# Autodesk Inventor assembly: Intake
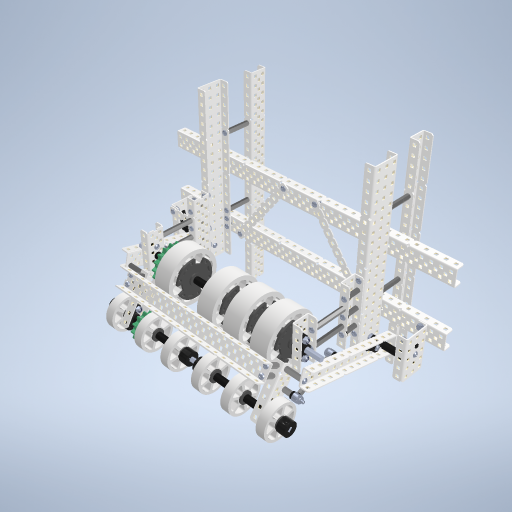
[picture p0: Inventor's stored thumbnail of the model, 512x512]
Saved by Autodesk Inventor 2023 (Build 270158000, 158)
## iProperties
Created: 2022-09-02
Part Number: Intake
Document SubType Name: Assembly
Designer: alex
Author: alex
## Documents named in this file (42)
- C:\Users\alex\Documents\GitHub\4067X_spin_up_cad\Mechanism\Intake.iam
- C:\Users\alex\Documents\GitHub\4067X_spin_up_cad\Library\Structure\Standoff\Standoff 1.00.ipt
- C:\Users\alex\Documents\GitHub\4067X_spin_up_cad\Library\Structure\Standoff.ipt
- C:\Users\alex\Documents\GitHub\4067X_spin_up_cad\Library\Structure\Hardware\Screw Steel - Star\SScrew Star Smooth .290.ipt
- C:\Users\alex\Documents\GitHub\4067X_spin_up_cad\Library\Structure\Hardware\Screw Steel - Star.ipt
- C:\Users\alex\Documents\GitHub\4067X_spin_up_cad\Library\Structure\Standoff\Standoff .50.ipt
- C:\Users\alex\Documents\GitHub\4067X_spin_up_cad\Library\Motion\Spacers\Spacer Nylon .375 OD.ipt
- C:\Users\alex\Documents\GitHub\4067X_spin_up_cad\Library\Structure\Hardware\Nut Keps.ipt
- C:\Users\alex\Documents\GitHub\4067X_spin_up_cad\Library\Motion\1-Post Bearing Flat Hex Retainer.ipt
- C:\Users\alex\Documents\GitHub\4067X_spin_up_cad\Library\Structure\Hardware\Screw Steel - Star\SScrew Star Smooth .375.ipt
- C:\Users\alex\Documents\GitHub\4067X_spin_up_cad\Library\Structure\Hardware\Nut Nylock.ipt
- C:\Users\alex\Documents\GitHub\4067X_spin_up_cad\Library\Structure\C-Channels\Aluminum 1x3x1\Alu C 1x3x1x20.ipt
- C:\Users\alex\Documents\GitHub\4067X_spin_up_cad\Library\Structure\C-Channels\Aluminum 1x3x1\Alu C 1x3x1x5.ipt
- C:\Users\alex\Documents\GitHub\4067X_spin_up_cad\Library\Structure\C-Channels\Aluminum 1x2x1\Alu C 1x2x1x35.ipt
- C:\Users\alex\Documents\GitHub\4067X_spin_up_cad\Library\Structure\Hardware\Screw Steel - Star\SScrew Star Smooth 2.500.ipt
- C:\Users\alex\Documents\GitHub\4067X_spin_up_cad\Library\Motion\Spacers\Spacer Nylon .375 OD\NSpacer .375 OD x .375.ipt
- C:\Users\alex\Documents\GitHub\4067X_spin_up_cad\Library\Motion\Spacers\Spacer Nylon .375 OD\NSpacer .375 OD x .500.ipt
- C:\Users\alex\Documents\GitHub\4067X_spin_up_cad\Library\Structure\C-Channels\Aluminum 1x2x1\Alu C 1x2x1x25.ipt
- C:\Users\alex\Documents\GitHub\4067X_spin_up_cad\Library\Structure\Hardware\Screw Steel - Star\SScrew Star Smooth .750.ipt
- C:\Users\alex\Documents\GitHub\4067X_spin_up_cad\Mechanism\FloatingIntake.iam
- C:\Users\alex\Documents\GitHub\4067X_spin_up_cad\Library\Motion\Spacers\Spacer Nylon .375 OD\NSpacer .375 OD x .250.ipt
- C:\Users\alex\Documents\GitHub\4067X_spin_up_cad\Library\Motion\Spacers\Washer Teflon\TWasher .375 OD x .06250.ipt
- C:\Users\alex\Documents\GitHub\4067X_spin_up_cad\Library\Motion\Spacers\Washer Teflon.ipt
- C:\Users\alex\Documents\GitHub\4067X_spin_up_cad\Library\Motion\Spacers\Washer Teflon\TWasher .375 OD x .04000.ipt
- C:\Users\alex\Documents\GitHub\4067X_spin_up_cad\Library\Structure\Plates\Aluminum\VEX Plates\Alu Plate VEX 1x11.ipt
- C:\Users\alex\Documents\GitHub\4067X_spin_up_cad\Library\Structure\Plates\Aluminum\VEX Plates\Alu Plate VEX 1x6.ipt
- C:\Users\alex\Documents\GitHub\4067X_spin_up_cad\Library\Structure\Standoff\Standoff 2.00.ipt
- C:\Users\alex\Documents\GitHub\4067X_spin_up_cad\Library\Structure\C-Channels\Aluminum 1x2x1\Alu C 1x2x1x5.ipt
- C:\Users\alex\Documents\GitHub\4067X_spin_up_cad\Library\Structure\C-Channels\Aluminum 1x2x1\Alu C 1x2x1x7.ipt
- C:\Users\alex\Documents\GitHub\4067X_spin_up_cad\Library\Structure\Standoff\Standoff .75.ipt
- C:\Users\alex\Documents\GitHub\4067X_spin_up_cad\Library\Motion\Spacers\Spacer Nylon .375 OD\NSpacer .375 OD x .125.ipt
- C:\Users\alex\Documents\GitHub\4067X_spin_up_cad\Library\Motion\Shaft HS\HS Bearing Flat.ipt
- C:\Users\alex\Documents\GitHub\4067X_spin_up_cad\Library\Structure\Hardware\Nut Thin Nylock.ipt
- C:\Users\alex\Documents\GitHub\4067X_spin_up_cad\Library\Structure\Hardware\Screw Steel - Star\SScrew Star Smooth .500.ipt
- C:\Users\alex\Documents\GitHub\4067X_spin_up_cad\Library\Motion\Shaft HS\Shaft HS\Shaft HS 12.0 in.ipt
- C:\Users\alex\Documents\GitHub\4067X_spin_up_cad\Library\Motion\Shaft HS\Shaft HS.ipt
- C:\Users\alex\Documents\GitHub\4067X_spin_up_cad\Library\Motion\Shaft HS\HS Spacer.ipt
- C:\Users\alex\Documents\GitHub\4067X_spin_up_cad\Library\3FlexWheel.iam
- C:\Users\alex\Documents\GitHub\4067X_spin_up_cad\Library\Motion\Shaft HS\HS Spacer\HSpacer .2500.ipt
- C:\Users\alex\Documents\GitHub\4067X_spin_up_cad\Library\Motion\Shaft HS\HS Spacer\HSpacer .5000.ipt
- C:\Users\alex\Documents\GitHub\4067X_spin_up_cad\Library\Motion\Sprockets\HS 18T Sprocket, No Insert.ipt
- C:\Users\alex\Documents\GitHub\4067X_spin_up_cad\Library\Motion\Shaft HS\HS Spacer\HSpacer .1250.ipt
## Components (148 placed, 35 different names)
1. Alu C 1x3x1x5:1 — Insert:107, Insert:108, Insert:120, Mate:15, Insert:145, Insert:230, Insert:244, Insert:245
2. Alu C 1x2x1x35:1 — Insert:107, Insert:108, Insert:150, Insert:151, Insert:218, Insert:219, Insert:236, Insert:237, Insert:252, Insert:253, Insert:277, Insert:278, Insert:285, Insert:286, Insert:304, Insert:305, Insert:309, Insert:313, Insert:314, Insert:317
3. Standoff 1.00:16 — Insert:110, Insert:287
4. Standoff .50:17 — Insert:110, Insert:125
5. Standoff 1.00:18 — Insert:288
6. Standoff .50:19 — Insert:124
7. 1-Post Bearing Flat Hex Retainer:2 — Insert:120, Mate:15, Insert:146
8. NSpacer .375 OD x .500:4 — Insert:122, Insert:294
9. NSpacer .375 OD x .500:5 — Insert:122, Insert:123
10. NSpacer .375 OD x .375:6 — Insert:123
11. Alu C 1x2x1x25:1 — Insert:124, Insert:125, Insert:239, Insert:240
12. Alu C 1x3x1x20:2 — Insert:252, Insert:253, Mate:35, Insert:254, Insert:255, Insert:260, Insert:263, Insert:267, Insert:268, Insert:275, Insert:276, Insert:283, Insert:284, Insert:342, Insert:343, Insert:344, Insert:350, Insert:351, Insert:352, Insert:353, Insert:354
13. Standoff 1.00:20 — Insert:260
14. Standoff .50:21 — Insert:133
15. Standoff 1.00:22 — Insert:344
16. Standoff .50:23 — Insert:132
17. Alu C 1x2x1x25:2 — Insert:132, Insert:133, Insert:227, Insert:243
18. NSpacer .375 OD x .500:8 — Insert:259
19. NSpacer .375 OD x .500:9
20. NSpacer .375 OD x .375:10
21. SScrew Star Smooth .375:34 — Insert:145
22. Nut Nylock:3 — Insert:146
23. Alu C 1x3x1x5:2 — Insert:150, Insert:151, Insert:217, Insert:220, Insert:221, Insert:330
24. 1-Post Bearing Flat Hex Retainer:4
25. SScrew Star Smooth .375:35
26. Nut Nylock:4
27. Nut Keps:12 — Insert:217
28. SScrew Star Smooth .290:52 — Insert:218
29. SScrew Star Smooth .290:53 — Insert:219
30. Nut Keps:13 — Insert:220
31. Nut Keps:14 — Insert:221
32. SScrew Star Smooth .750:57 — Insert:227
33. Nut Keps:17 — Insert:230
34. SScrew Star Smooth .290:62 — Insert:236
35. SScrew Star Smooth .290:63 — Insert:237
36. SScrew Star Smooth .750:65 — Insert:239
37. SScrew Star Smooth .750:66 — Insert:240
38. SScrew Star Smooth .750:69 — Insert:243
39. Nut Keps:21 — Insert:244
40. Nut Keps:22 — Insert:245
41. FloatingIntake:1 [sub-assembly] — Mate:35, Mate:36, Insert:259, Mate:37, Insert:294, Rotation:1
42. SScrew Star Smooth 2.500:75 — Insert:254, Mate:36
43. Nut Keps:23 — Insert:255, Insert:256
44. NSpacer .375 OD x .250:11 — Insert:256, Insert:257
45. TWasher .375 OD x .06250:1 — Insert:257, Insert:258
46. TWasher .375 OD x .04000:2 — Insert:258
47. SScrew Star Smooth .290:78 — Insert:263
48. Alu C 1x2x1x35:2 — Insert:267, Insert:268, Insert:308, Insert:312, Insert:315, Insert:316
49. SScrew Star Smooth .290:82 — Insert:275
50. SScrew Star Smooth .290:83 — Insert:276
51. Nut Keps:28 — Insert:277
52. Nut Keps:29 — Insert:278
53. Nut Keps:30 — Insert:283
54. SScrew Star Smooth .290:86 — Insert:284
55. Alu C 1x3x1x20:3 — Insert:285, Insert:286, Insert:287, Insert:288, Mate:37, Insert:289, Insert:293, Insert:300, Insert:301, Insert:302, Insert:303, Insert:380, Insert:385
56. SScrew Star Smooth 2.500:87 — Insert:289
57. Nut Keps:31 — Insert:293
58. NSpacer .375 OD x .250:12
59. TWasher .375 OD x .06250:3
60. TWasher .375 OD x .04000:4
61. SScrew Star Smooth .290:90 — Insert:300
62. SScrew Star Smooth .290:91 — Insert:301
63. SScrew Star Smooth .290:92 — Insert:302
64. SScrew Star Smooth .290:93 — Insert:303
65. Nut Keps:33 — Insert:304
66. Nut Keps:34 — Insert:305
67. Alu Plate VEX 1x11:2 — Insert:308, Insert:309
68. SScrew Star Smooth .290:94
69. SScrew Star Smooth .290:95
70. Alu Plate VEX 1x11:3 — Insert:312, Insert:313
71. SScrew Star Smooth .290:96
72. SScrew Star Smooth .290:97
73. Nut Keps:35 — Insert:314
74. Nut Keps:36 — Insert:315
75. Nut Keps:37 — Insert:316
76. Nut Keps:38 — Insert:317
77. Alu C 1x2x1x5:2 — Insert:334, Insert:335, Insert:338, Insert:339, Insert:387, Insert:388, Mate:38, Insert:389, Flush:1, Mate:61
78. TWasher .375 OD x .06250:5 — Insert:330, Insert:331
79. Alu Plate VEX 1x6:3 — Insert:331, Insert:340, Insert:341
80. Standoff 2.00:27 — Insert:334, Insert:382
81. Standoff 2.00:28 — Insert:335, Insert:381
82. SScrew Star Smooth .290:102 — Insert:338
83. SScrew Star Smooth .290:103 — Insert:339
84. SScrew Star Smooth .375:104 — Insert:340
85. SScrew Star Smooth .375:105 — Insert:341
86. Alu C 1x2x1x7:1 — Insert:342, Insert:343, Insert:345, Insert:346, Insert:347, Insert:348, Insert:349, Insert:358, Insert:359, Insert:360, Insert:361, Insert:362, Insert:381, Insert:382
87. SScrew Star Smooth .290:106 — Insert:345
88. SScrew Star Smooth .290:107 — Insert:346
89. Standoff .75:29 — Insert:347, Insert:355
90. Standoff .75:30 — Insert:348, Insert:356
91. Standoff .75:31 — Insert:349, Insert:357
92. SScrew Star Smooth .290:108 — Insert:350
93. SScrew Star Smooth .290:109 — Insert:351
94. SScrew Star Smooth .290:110 — Insert:352
95. Nut Keps:39 — Insert:353
96. Nut Keps:40 — Insert:354
97. NSpacer .375 OD x .125:13 — Insert:355
98. NSpacer .375 OD x .125:14 — Insert:356
99. NSpacer .375 OD x .125:15 — Insert:357
100. SScrew Star Smooth .375:111 — Insert:358
101. SScrew Star Smooth .375:112 — Insert:359
102. SScrew Star Smooth .375:113 — Insert:360
103. SScrew Star Smooth .290:114 — Insert:361
104. SScrew Star Smooth .290:115 — Insert:362
105. Alu C 1x2x1x5:3 — Insert:393, Mate:39, Insert:394, Insert:395, Mate:45
106. Standoff 2.00:32 — Insert:384
107. Standoff 2.00:33 — Insert:383
108. SScrew Star Smooth .290:116
109. SScrew Star Smooth .290:117
110. Alu C 1x2x1x7:2 — Insert:380, Insert:383, Insert:384, Insert:385
111. SScrew Star Smooth .290:118
112. SScrew Star Smooth .290:119
113. Standoff .75:34
114. Standoff .75:35
115. Standoff .75:36
116. NSpacer .375 OD x .125:16
117. NSpacer .375 OD x .125:17
118. NSpacer .375 OD x .125:18
119. SScrew Star Smooth .375:120
120. SScrew Star Smooth .375:121
121. SScrew Star Smooth .375:122
122. SScrew Star Smooth .290:123
123. SScrew Star Smooth .290:124
124. HS Bearing Flat:1 — Insert:387, Mate:38, Insert:390, Mate:40
125. Nut Thin Nylock:1
126. SScrew Star Smooth .500:125 — Insert:388
127. SScrew Star Smooth .500:126 — Insert:389
128. Nut Thin Nylock:2 — Insert:390
129. HS Bearing Flat:2 — Insert:393, Mate:39
130. Nut Thin Nylock:3
131. Nut Thin Nylock:4
132. SScrew Star Smooth .500:127 — Insert:394
133. SScrew Star Smooth .500:128 — Insert:395
134. Shaft HS 12.0 in:1 — Mate:40, Flush:1, Mate:43, Angle:1, Mate:44, Angle:2, Mate:47, Mate:50, Mate:51, Mate:53, Angle:3, Mate:55, Mate:57, Angle:4, Mate:58, Angle:5, Mate:60, Mate:62
135. 3FlexWheel:1 [sub-assembly] — Mate:43, Angle:1, Mate:46, Mate:48
136. HSpacer .2500:1 — Mate:44, Mate:45, Mate:46
137. 3FlexWheel:2 [sub-assembly] — Angle:2, Mate:49, Mate:50, Mate:52
138. HSpacer .2500:2 — Mate:47, Mate:48, Mate:49
139. HSpacer .2500:3 — Mate:51, Mate:52, Mate:54
140. 3FlexWheel:3 [sub-assembly] — Mate:53, Angle:3, Mate:54, Mate:56
141. 3FlexWheel:4 [sub-assembly] — Mate:58, Angle:5, Mate:59, Mate:64
142. HSpacer .5000:4 — Mate:55, Mate:56, Insert:397
143. HS 18T Sprocket, No Insert:1 — Mate:57, Angle:4, Rotation:1, Mate:59
144. HSpacer .5000:5 — Mate:60, Mate:61, Mate:63
145. HSpacer .2500:6 — Mate:62, Mate:63, Insert:399
146. HSpacer .5000:8 — Insert:397, Insert:398
147. HSpacer .5000:9 — Insert:398, Mate:64
148. HSpacer .1250:10 — Insert:399
## Relationships (184: Insert 147, Mate 30, Angle 5, Flush 1, RelateRotation 1)
- Insert:107: Alu C 1x3x1x5:1 ↔ Alu C 1x2x1x35:1
- Insert:108: Alu C 1x3x1x5:1 ↔ Alu C 1x2x1x35:1
- Insert:110: Standoff 1.00:16 ↔ Standoff .50:17
- [Insert]: Standoff 1.00:18 ↔ Standoff .50:19
- Insert:120: Alu C 1x3x1x5:1 ↔ 1-Post Bearing Flat Hex Retainer:2
- Mate:15: Alu C 1x3x1x5:1 ↔ 1-Post Bearing Flat Hex Retainer:2
- Insert:122: NSpacer .375 OD x .500:4 ↔ NSpacer .375 OD x .500:5
- Insert:123: NSpacer .375 OD x .500:5 ↔ NSpacer .375 OD x .375:6
- Insert:124: Standoff .50:19 ↔ Alu C 1x2x1x25:1
- Insert:125: Standoff .50:17 ↔ Alu C 1x2x1x25:1
- [Insert]: Standoff 1.00:20 ↔ Standoff .50:21
- [Insert]: Standoff 1.00:22 ↔ Standoff .50:23
- Insert:132: Standoff .50:23 ↔ Alu C 1x2x1x25:2
- Insert:133: Standoff .50:21 ↔ Alu C 1x2x1x25:2
- [Insert]: NSpacer .375 OD x .500:8 ↔ NSpacer .375 OD x .500:9
- [Insert]: NSpacer .375 OD x .500:9 ↔ NSpacer .375 OD x .375:10
- Insert:145: Alu C 1x3x1x5:1 ↔ SScrew Star Smooth .375:34
- Insert:146: 1-Post Bearing Flat Hex Retainer:2 ↔ Nut Nylock:3
- [Insert]: Alu C 1x3x1x5:2 ↔ 1-Post Bearing Flat Hex Retainer:4
- [Mate]: Alu C 1x3x1x5:2 ↔ 1-Post Bearing Flat Hex Retainer:4
- [Insert]: Alu C 1x3x1x5:2 ↔ SScrew Star Smooth .375:35
- [Insert]: 1-Post Bearing Flat Hex Retainer:4 ↔ Nut Nylock:4
- Insert:150: Alu C 1x2x1x35:1 ↔ Alu C 1x3x1x5:2
- Insert:151: Alu C 1x2x1x35:1 ↔ Alu C 1x3x1x5:2
- Insert:217: Alu C 1x3x1x5:2 ↔ Nut Keps:12
- Insert:218: Alu C 1x2x1x35:1 ↔ SScrew Star Smooth .290:52
- Insert:219: Alu C 1x2x1x35:1 ↔ SScrew Star Smooth .290:53
- Insert:220: Alu C 1x3x1x5:2 ↔ Nut Keps:13
- Insert:221: Alu C 1x3x1x5:2 ↔ Nut Keps:14
- Insert:227: Alu C 1x2x1x25:2 ↔ SScrew Star Smooth .750:57
- Insert:230: Alu C 1x3x1x5:1 ↔ Nut Keps:17
- Insert:236: Alu C 1x2x1x35:1 ↔ SScrew Star Smooth .290:62
- Insert:237: Alu C 1x2x1x35:1 ↔ SScrew Star Smooth .290:63
- Insert:239: Alu C 1x2x1x25:1 ↔ SScrew Star Smooth .750:65
- Insert:240: Alu C 1x2x1x25:1 ↔ SScrew Star Smooth .750:66
- Insert:243: Alu C 1x2x1x25:2 ↔ SScrew Star Smooth .750:69
- Insert:244: Alu C 1x3x1x5:1 ↔ Nut Keps:21
- Insert:245: Alu C 1x3x1x5:1 ↔ Nut Keps:22
- Insert:252: Alu C 1x2x1x35:1 ↔ Alu C 1x3x1x20:2
- Insert:253: Alu C 1x2x1x35:1 ↔ Alu C 1x3x1x20:2
- Mate:35 (12.7 mm): Alu C 1x3x1x20:2 ↔ FloatingIntake:1
- Insert:254: Alu C 1x3x1x20:2 ↔ SScrew Star Smooth 2.500:75
- Insert:255: Alu C 1x3x1x20:2 ↔ Nut Keps:23
- Mate:36: FloatingIntake:1 ↔ SScrew Star Smooth 2.500:75
- Insert:256: Nut Keps:23 ↔ NSpacer .375 OD x .250:11
- Insert:257: NSpacer .375 OD x .250:11 ↔ TWasher .375 OD x .06250:1
- Insert:258: TWasher .375 OD x .06250:1 ↔ TWasher .375 OD x .04000:2
- Insert:259: NSpacer .375 OD x .500:8 ↔ FloatingIntake:1
- Insert:260: Alu C 1x3x1x20:2 ↔ Standoff 1.00:20
- Insert:263: Alu C 1x3x1x20:2 ↔ SScrew Star Smooth .290:78
- Insert:267: Alu C 1x3x1x20:2 ↔ Alu C 1x2x1x35:2
- Insert:268: Alu C 1x3x1x20:2 ↔ Alu C 1x2x1x35:2
- Insert:275: Alu C 1x3x1x20:2 ↔ SScrew Star Smooth .290:82
- Insert:276: Alu C 1x3x1x20:2 ↔ SScrew Star Smooth .290:83
- Insert:277: Alu C 1x2x1x35:1 ↔ Nut Keps:28
- Insert:278: Alu C 1x2x1x35:1 ↔ Nut Keps:29
- Insert:283: Alu C 1x3x1x20:2 ↔ Nut Keps:30
- Insert:284: Alu C 1x3x1x20:2 ↔ SScrew Star Smooth .290:86
- Insert:285: Alu C 1x2x1x35:1 ↔ Alu C 1x3x1x20:3
- Insert:286: Alu C 1x2x1x35:1 ↔ Alu C 1x3x1x20:3
- Insert:287: Standoff 1.00:16 ↔ Alu C 1x3x1x20:3
- Insert:288: Standoff 1.00:18 ↔ Alu C 1x3x1x20:3
- Mate:37 (12.7 mm): FloatingIntake:1 ↔ Alu C 1x3x1x20:3
- Insert:289: Alu C 1x3x1x20:3 ↔ SScrew Star Smooth 2.500:87
- [Insert]: Nut Keps:31 ↔ NSpacer .375 OD x .250:12
- [Insert]: NSpacer .375 OD x .250:12 ↔ TWasher .375 OD x .06250:3
- [Insert]: TWasher .375 OD x .06250:3 ↔ TWasher .375 OD x .04000:4
- Insert:293: Alu C 1x3x1x20:3 ↔ Nut Keps:31
- Insert:294: NSpacer .375 OD x .500:4 ↔ FloatingIntake:1
- Insert:300: Alu C 1x3x1x20:3 ↔ SScrew Star Smooth .290:90
- Insert:301: Alu C 1x3x1x20:3 ↔ SScrew Star Smooth .290:91
- Insert:302: Alu C 1x3x1x20:3 ↔ SScrew Star Smooth .290:92
- Insert:303: Alu C 1x3x1x20:3 ↔ SScrew Star Smooth .290:93
- Insert:304: Alu C 1x2x1x35:1 ↔ Nut Keps:33
- Insert:305: Alu C 1x2x1x35:1 ↔ Nut Keps:34
- [Insert]: Alu Plate VEX 1x11:2 ↔ SScrew Star Smooth .290:94
- [Insert]: Alu Plate VEX 1x11:2 ↔ SScrew Star Smooth .290:95
- Insert:308: Alu C 1x2x1x35:2 ↔ Alu Plate VEX 1x11:2
- Insert:309: Alu C 1x2x1x35:1 ↔ Alu Plate VEX 1x11:2
- [Insert]: Alu Plate VEX 1x11:3 ↔ SScrew Star Smooth .290:96
- [Insert]: Alu Plate VEX 1x11:3 ↔ SScrew Star Smooth .290:97
- Insert:312: Alu C 1x2x1x35:2 ↔ Alu Plate VEX 1x11:3
- Insert:313: Alu C 1x2x1x35:1 ↔ Alu Plate VEX 1x11:3
- Insert:314: Alu C 1x2x1x35:1 ↔ Nut Keps:35
- Insert:315: Alu C 1x2x1x35:2 ↔ Nut Keps:36
- Insert:316: Alu C 1x2x1x35:2 ↔ Nut Keps:37
- Insert:317: Alu C 1x2x1x35:1 ↔ Nut Keps:38
- Insert:330: Alu C 1x3x1x5:2 ↔ TWasher .375 OD x .06250:5
- Insert:331: TWasher .375 OD x .06250:5 ↔ Alu Plate VEX 1x6:3
- Insert:334: Alu C 1x2x1x5:2 ↔ Standoff 2.00:27
- Insert:335: Alu C 1x2x1x5:2 ↔ Standoff 2.00:28
- Insert:338: Alu C 1x2x1x5:2 ↔ SScrew Star Smooth .290:102
- Insert:339: Alu C 1x2x1x5:2 ↔ SScrew Star Smooth .290:103
- Insert:340: Alu Plate VEX 1x6:3 ↔ SScrew Star Smooth .375:104
- Insert:341: Alu Plate VEX 1x6:3 ↔ SScrew Star Smooth .375:105
- Insert:342: Alu C 1x3x1x20:2 ↔ Alu C 1x2x1x7:1
- Insert:343: Alu C 1x3x1x20:2 ↔ Alu C 1x2x1x7:1
- Insert:344: Alu C 1x3x1x20:2 ↔ Standoff 1.00:22
- Insert:345: Alu C 1x2x1x7:1 ↔ SScrew Star Smooth .290:106
- Insert:346: Alu C 1x2x1x7:1 ↔ SScrew Star Smooth .290:107
- Insert:347: Alu C 1x2x1x7:1 ↔ Standoff .75:29
- Insert:348: Alu C 1x2x1x7:1 ↔ Standoff .75:30
- Insert:349: Alu C 1x2x1x7:1 ↔ Standoff .75:31
- Insert:350: Alu C 1x3x1x20:2 ↔ SScrew Star Smooth .290:108
- Insert:351: Alu C 1x3x1x20:2 ↔ SScrew Star Smooth .290:109
- Insert:352: Alu C 1x3x1x20:2 ↔ SScrew Star Smooth .290:110
- Insert:353: Alu C 1x3x1x20:2 ↔ Nut Keps:39
- Insert:354: Alu C 1x3x1x20:2 ↔ Nut Keps:40
- Insert:355: Standoff .75:29 ↔ NSpacer .375 OD x .125:13
- Insert:356: Standoff .75:30 ↔ NSpacer .375 OD x .125:14
- Insert:357: Standoff .75:31 ↔ NSpacer .375 OD x .125:15
- Insert:358: Alu C 1x2x1x7:1 ↔ SScrew Star Smooth .375:111
- Insert:359: Alu C 1x2x1x7:1 ↔ SScrew Star Smooth .375:112
- Insert:360: Alu C 1x2x1x7:1 ↔ SScrew Star Smooth .375:113
- Insert:361: Alu C 1x2x1x7:1 ↔ SScrew Star Smooth .290:114
- Insert:362: Alu C 1x2x1x7:1 ↔ SScrew Star Smooth .290:115
- [Insert]: Alu C 1x2x1x5:3 ↔ Standoff 2.00:32
- [Insert]: Alu C 1x2x1x5:3 ↔ Standoff 2.00:33
- [Insert]: Alu C 1x2x1x5:3 ↔ SScrew Star Smooth .290:116
- [Insert]: Alu C 1x2x1x5:3 ↔ SScrew Star Smooth .290:117
- [Insert]: Alu C 1x2x1x7:2 ↔ SScrew Star Smooth .290:118
- [Insert]: Alu C 1x2x1x7:2 ↔ SScrew Star Smooth .290:119
- [Insert]: Alu C 1x2x1x7:2 ↔ Standoff .75:34
- [Insert]: Alu C 1x2x1x7:2 ↔ Standoff .75:35
- [Insert]: Alu C 1x2x1x7:2 ↔ Standoff .75:36
- [Insert]: Standoff .75:34 ↔ NSpacer .375 OD x .125:16
- [Insert]: Standoff .75:35 ↔ NSpacer .375 OD x .125:17
- [Insert]: Standoff .75:36 ↔ NSpacer .375 OD x .125:18
- [Insert]: Alu C 1x2x1x7:2 ↔ SScrew Star Smooth .375:120
- [Insert]: Alu C 1x2x1x7:2 ↔ SScrew Star Smooth .375:121
- [Insert]: Alu C 1x2x1x7:2 ↔ SScrew Star Smooth .375:122
- [Insert]: Alu C 1x2x1x7:2 ↔ SScrew Star Smooth .290:123
- [Insert]: Alu C 1x2x1x7:2 ↔ SScrew Star Smooth .290:124
- Insert:380: Alu C 1x3x1x20:3 ↔ Alu C 1x2x1x7:2
- Insert:381: Standoff 2.00:28 ↔ Alu C 1x2x1x7:1
- Insert:382: Standoff 2.00:27 ↔ Alu C 1x2x1x7:1
- Insert:383: Standoff 2.00:33 ↔ Alu C 1x2x1x7:2
- Insert:384: Standoff 2.00:32 ↔ Alu C 1x2x1x7:2
- Insert:385: Alu C 1x3x1x20:3 ↔ Alu C 1x2x1x7:2
- [Insert]: HS Bearing Flat:1 ↔ Nut Thin Nylock:1
- Insert:387: Alu C 1x2x1x5:2 ↔ HS Bearing Flat:1
- Insert:388: Alu C 1x2x1x5:2 ↔ SScrew Star Smooth .500:125
- Mate:38: Alu C 1x2x1x5:2 ↔ HS Bearing Flat:1
- Insert:389: Alu C 1x2x1x5:2 ↔ SScrew Star Smooth .500:126
- Insert:390: HS Bearing Flat:1 ↔ Nut Thin Nylock:2
- [Insert]: HS Bearing Flat:2 ↔ Nut Thin Nylock:3
- [Insert]: HS Bearing Flat:2 ↔ Nut Thin Nylock:4
- Insert:393: Alu C 1x2x1x5:3 ↔ HS Bearing Flat:2
- Mate:39: Alu C 1x2x1x5:3 ↔ HS Bearing Flat:2
- Insert:394: Alu C 1x2x1x5:3 ↔ SScrew Star Smooth .500:127
- Insert:395: Alu C 1x2x1x5:3 ↔ SScrew Star Smooth .500:128
- Mate:40: HS Bearing Flat:1 ↔ Shaft HS 12.0 in:1
- Flush:1 (-31.4198 mm): Alu C 1x2x1x5:2 ↔ Shaft HS 12.0 in:1
- Mate:43: Shaft HS 12.0 in:1 ↔ 3FlexWheel:1
- Angle:1 (0 deg): Shaft HS 12.0 in:1 ↔ 3FlexWheel:1
- Mate:44: Shaft HS 12.0 in:1 ↔ HSpacer .2500:1
- Mate:45: Alu C 1x2x1x5:3 ↔ HSpacer .2500:1
- Mate:46: 3FlexWheel:1 ↔ HSpacer .2500:1
- Angle:2 (0 deg): Shaft HS 12.0 in:1 ↔ 3FlexWheel:2
- Mate:47: Shaft HS 12.0 in:1 ↔ HSpacer .2500:2
- Mate:48: 3FlexWheel:1 ↔ HSpacer .2500:2
- Mate:49: 3FlexWheel:2 ↔ HSpacer .2500:2
- Mate:50: Shaft HS 12.0 in:1 ↔ 3FlexWheel:2
- Mate:51: Shaft HS 12.0 in:1 ↔ HSpacer .2500:3
- Mate:52: 3FlexWheel:2 ↔ HSpacer .2500:3
- Mate:53: Shaft HS 12.0 in:1 ↔ 3FlexWheel:3
- Angle:3 (0 deg): Shaft HS 12.0 in:1 ↔ 3FlexWheel:3
- Mate:54: HSpacer .2500:3 ↔ 3FlexWheel:3
- Mate:55: Shaft HS 12.0 in:1 ↔ HSpacer .5000:4
- Mate:56: 3FlexWheel:3 ↔ HSpacer .5000:4
- Mate:57: Shaft HS 12.0 in:1 ↔ HS 18T Sprocket, No Insert:1
- Angle:4 (0 deg): Shaft HS 12.0 in:1 ↔ HS 18T Sprocket, No Insert:1
- Rotation:1 [RelateRotation] (0.6667 ul): FloatingIntake:1 ↔ HS 18T Sprocket, No Insert:1
- Mate:58: Shaft HS 12.0 in:1 ↔ 3FlexWheel:4
- Angle:5 (0 deg): Shaft HS 12.0 in:1 ↔ 3FlexWheel:4
- Mate:59: 3FlexWheel:4 ↔ HS 18T Sprocket, No Insert:1
- Mate:60: Shaft HS 12.0 in:1 ↔ HSpacer .5000:5
- Mate:61: Alu C 1x2x1x5:2 ↔ HSpacer .5000:5
- Mate:62: Shaft HS 12.0 in:1 ↔ HSpacer .2500:6
- Mate:63: HSpacer .5000:5 ↔ HSpacer .2500:6
- Insert:397: HSpacer .5000:4 ↔ HSpacer .5000:8
- Insert:398: HSpacer .5000:8 ↔ HSpacer .5000:9
- Mate:64: 3FlexWheel:4 ↔ HSpacer .5000:9
- Insert:399: HSpacer .2500:6 ↔ HSpacer .1250:10
## Named parameters: d171_d169 = 0 mm, d195_d169 = 0 mm, d197_d195_d169 = 0 mm, d210_d188 = 0 mm, d211_d189 = 0 mm, d215_d185 = 0 mm, d216_d186 = 0 mm, d217_d213 = 0 mm, d218_d214 = 0 mm, d407_d369 = 0 mm, d408_d370 = 0 mm, d409_d371 = 0 mm, d423_d386 = 0 mm, d424_d387 = 0 mm, d427_d423_d386 = 0 mm, d428_d424_d387 = 0 mm, d492_d477 = 0 mm, d493_d478 = 0 mm, d494_d484 = 0 mm, d495_d485 = 0 mm, d496_d486 = 0 mm, d497_d487 = 0 mm, d498_d488 = 0 mm, d499_d489 = 0 mm, d500_d490 = 0 mm, d501_d491 = 0 mm, d502_d463 = 0 mm, d503_d464 = 0 mm, d504_d467 = 0 mm, d505_d468 = 0 mm, d506_d474 = 0 mm, d507_d475 = 0 mm, d508_d476 = 0 mm, d253_d244 = 0 mm, d521_d253_d244 = 0 mm, d522_d520 = 0 mm
